# Autodesk Inventor assembly: ElvShaft
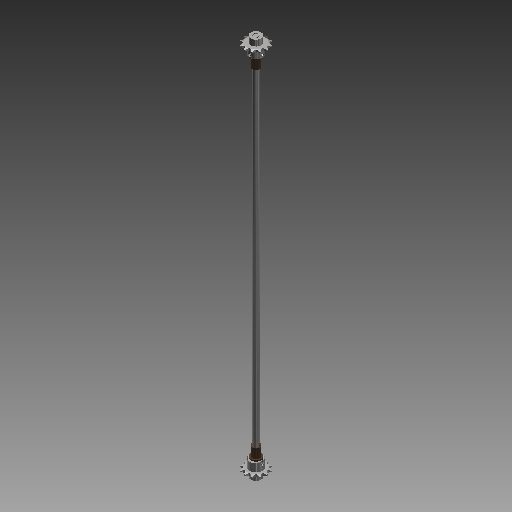
[picture p0: Inventor's stored thumbnail of the model, 512x512]
Saved by Autodesk Inventor 2019 (Build 230136000, 136)
## iProperties
Created: 2019-01-10
Part Number: ElvShaft
Document SubType Name: Assembly
Designer: james
Mass: 179.45 g
Surface Area: 167.573 cm^2
Volume: 22.4285 cm^3
Density: 8.00099 g/cm^3
Author: james
## Documents named in this file (5)
- F:\JimsDesign\2019CHS4089\ElvShaft.iam
- F:\JimsDesign\Library\McMaster\1327K670_MINIATURE 12L14 DRIVE STEEL SHAFT.ipt
- F:\JimsDesign\Library\McMaster\9414T600_SET SCREW SHAFT COLLAR.ipt
- F:\JimsDesign\Library\McMaster\2737T101_FINISHED-BORE SPROCKET FOR ANSI ROLLER CHAIN.ipt
- F:\JimsDesign\Library\McMaster\6338K413_OIL-EMBEDDED FLANGED SLEEVE BEARING.ipt
## Components (7 placed, 4 different names)
1. 1327K670_MINIATURE 12L14 DRIVE STEEL SHAFT:1 — Mate:1, Flush:1, Mate:2, Flush:2, Mate:3, Mate:5, Mate:7, Mate:9
2. 9414T600_SET SCREW SHAFT COLLAR:1 — Mate:1, Flush:1, Mate:6
3. 9414T600_SET SCREW SHAFT COLLAR:2 — Mate:2, Flush:2, Mate:4
4. 2737T101_FINISHED-BORE SPROCKET FOR ANSI ROLLER CHAIN:1 — Mate:3, Mate:4, Mate:8
5. 2737T101_FINISHED-BORE SPROCKET FOR ANSI ROLLER CHAIN:2 — Mate:5, Mate:6, Mate:10
6. 6338K413_OIL-EMBEDDED FLANGED SLEEVE BEARING:1 — Mate:9, Mate:10
7. 6338K413_OIL-EMBEDDED FLANGED SLEEVE BEARING:2 — Mate:7, Mate:8
## Relationships (12: Mate 10, Flush 2)
- Mate:1: 1327K670_MINIATURE 12L14 DRIVE STEEL SHAFT:1 ↔ 9414T600_SET SCREW SHAFT COLLAR:1
- Flush:1: 1327K670_MINIATURE 12L14 DRIVE STEEL SHAFT:1 ↔ 9414T600_SET SCREW SHAFT COLLAR:1
- Mate:2: 1327K670_MINIATURE 12L14 DRIVE STEEL SHAFT:1 ↔ 9414T600_SET SCREW SHAFT COLLAR:2
- Flush:2: 1327K670_MINIATURE 12L14 DRIVE STEEL SHAFT:1 ↔ 9414T600_SET SCREW SHAFT COLLAR:2
- Mate:3: 1327K670_MINIATURE 12L14 DRIVE STEEL SHAFT:1 ↔ 2737T101_FINISHED-BORE SPROCKET FOR ANSI ROLLER CHAIN:1
- Mate:4: 9414T600_SET SCREW SHAFT COLLAR:2 ↔ 2737T101_FINISHED-BORE SPROCKET FOR ANSI ROLLER CHAIN:1
- Mate:5: 1327K670_MINIATURE 12L14 DRIVE STEEL SHAFT:1 ↔ 2737T101_FINISHED-BORE SPROCKET FOR ANSI ROLLER CHAIN:2
- Mate:6: 9414T600_SET SCREW SHAFT COLLAR:1 ↔ 2737T101_FINISHED-BORE SPROCKET FOR ANSI ROLLER CHAIN:2
- Mate:7: 1327K670_MINIATURE 12L14 DRIVE STEEL SHAFT:1 ↔ 6338K413_OIL-EMBEDDED FLANGED SLEEVE BEARING:2
- Mate:8: 2737T101_FINISHED-BORE SPROCKET FOR ANSI ROLLER CHAIN:1 ↔ 6338K413_OIL-EMBEDDED FLANGED SLEEVE BEARING:2
- Mate:9: 1327K670_MINIATURE 12L14 DRIVE STEEL SHAFT:1 ↔ 6338K413_OIL-EMBEDDED FLANGED SLEEVE BEARING:1
- Mate:10: 2737T101_FINISHED-BORE SPROCKET FOR ANSI ROLLER CHAIN:2 ↔ 6338K413_OIL-EMBEDDED FLANGED SLEEVE BEARING:1
